# Autodesk Inventor assembly: Ceiling Comp 1 Centered Division
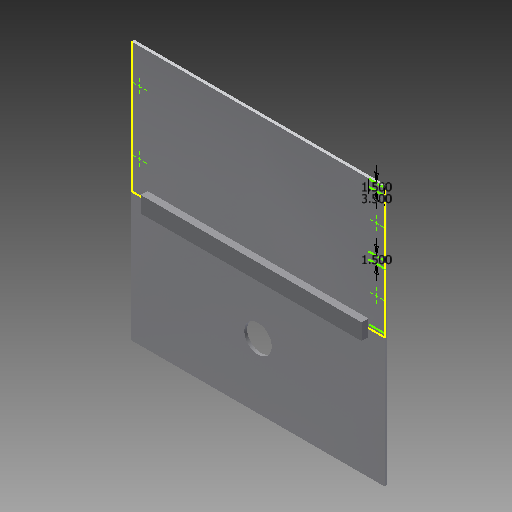
[picture p0: Inventor's stored thumbnail of the model, 512x512]
Saved by Autodesk Inventor 2017 (Build 210142000, 142)
## iProperties
Created: 2017-05-30
Part Number: Ceiling Comp 1 Centered Division
Document SubType Name: Assembly
Designer: cas7
Author: cas7
## Documents named in this file (4)
- C:\Users\Public\Documents\Autodesk\.desktop-connect\.docstore\guided-tutorial-plugin\INVNTOR\Compartment Modeling\Ceiling Comp 1 Centered Division.iam
- C:\Users\Public\Documents\Autodesk\.desktop-connect\.docstore\guided-tutorial-plugin\INVNTOR\Compartment Modeling\Half Ceiling Hole.ipt
- C:\Users\Public\Documents\Autodesk\.desktop-connect\.docstore\guided-tutorial-plugin\INVNTOR\2017\ENU\446352093014866114\TutorialModelPath\Half Ceiling Model 2.ipt
- C:\Users\Public\Documents\Autodesk\.desktop-connect\.docstore\guided-tutorial-plugin\INVNTOR\Compartment Modeling\48in 2x4.ipt
## Components (3 placed, 3 different names)
1. Half Ceiling Hole:1 — Mate:1, Mate:2, Mate:6
2. Half Ceiling Model 2:1 — Mate:1, Mate:2, Mate:3, Mate:4, Mate:5
3. 4ft 2x4:1 — Mate:3, Mate:4, Mate:5, Mate:6
## Relationships (6: Mate 6)
- Mate:1: Half Ceiling Hole:1 ↔ Half Ceiling Model 2:1
- Mate:2: Half Ceiling Hole:1 ↔ Half Ceiling Model 2:1
- Mate:3 (88.9 mm): Half Ceiling Model 2:1 ↔ 4ft 2x4:1
- Mate:4 (88.9 mm): Half Ceiling Model 2:1 ↔ 4ft 2x4:1
- Mate:5 (44.45 mm): Half Ceiling Model 2:1 ↔ 4ft 2x4:1
- Mate:6 (44.45 mm): Half Ceiling Hole:1 ↔ 4ft 2x4:1
